# Autodesk Inventor assembly: Ring1_Assembly_JacobMorgan_030415_pd3.ipt
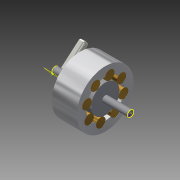
[picture p0: Inventor's stored thumbnail of the model, 180x180]
Saved by Autodesk Inventor 2015 (Build 190159000, 159)
## iProperties
Created: 2015-03-04
Part Number: Ring1_Assembly_JacobMorgan_030415_pd3.ipt
Document SubType Name: Assembly
Designer: WASHHSST
Author: WASHHSST
## Documents named in this file (6)
- E:\Ring1_Assembly_JacobMorgan_030415_pd3.ipt.iam
- E:\Ring1_NewDimensions_JacobMorgan_030215_pd3.ipt
- E:\Ring1_Center_JacobMorgan_030415_pd3.ipt
- E:\Ring1_Roller_JacobMorgan_030315_pd3.ipt
- E:\ring1_arm_JacobMorgan_030515_pd3.ipt
- E:\ring1_rollerFace_JacobMorgan_030515_pd3.ipt
## Components (19 placed, 5 different names)
1. Ring1_NewDimensions_JacobMorgan_030215_pd3:1 — Flush:1, Flush:2, Tangent:1, Flush:3, Flush:4, Flush:5, Flush:6, Flush:7, Flush:8, Flush:9, Tangent:2, Tangent:3, Tangent:4, Tangent:5, Tangent:6, Tangent:7, Tangent:8, Flush:10, Flush:11
2. Ring1_Center_JacobMorgan_030415_pd3:1 — Flush:1, Flush:2, Tangent:1, Tangent:12, Tangent:32, Tangent:33, Mate:9, Rotation:7
3. Ring1_Center_JacobMorgan_030415_pd3:2 — Flush:3, Tangent:4, Tangent:18, Tangent:26, Tangent:27, Mate:6, Rotation:2
4. Ring1_Center_JacobMorgan_030415_pd3:3 — Flush:4, Tangent:2, Tangent:10, Tangent:20, Tangent:22, Tangent:23, Mate:4, Rotation:6
5. Ring1_Center_JacobMorgan_030415_pd3:4 — Flush:5, Tangent:3, Tangent:9, Tangent:19, Rotation:1, Tangent:24, Tangent:25, Mate:5
6. Ring1_Center_JacobMorgan_030415_pd3:5 — Flush:6, Tangent:5, Tangent:17, Rotation:3, Tangent:30, Tangent:31, Mate:8
7. Ring1_Center_JacobMorgan_030415_pd3:6 — Flush:7, Tangent:8, Tangent:13, Tangent:34, Tangent:35, Mate:10, Rotation:8
8. Ring1_Center_JacobMorgan_030415_pd3:7 — Flush:8, Tangent:6, Tangent:16, Tangent:28, Tangent:29, Mate:7, Rotation:4
9. Ring1_Center_JacobMorgan_030415_pd3:8 — Flush:9, Tangent:7, Tangent:11, Flush:11, Tangent:14, Tangent:15, Tangent:36, Tangent:37, Mate:11, Rotation:5
10. Ring1_Roller_JacobMorgan_030315_pd3:1 — Flush:10, Tangent:9, Tangent:10, Tangent:11, Tangent:12, Tangent:13, Tangent:14, Tangent:15, Tangent:16, Tangent:17, Tangent:18, Tangent:19, Tangent:20, Mate:1, Mate:2, Mate:3, Tangent:21, Rotation:1, Rotation:2, Rotation:3, Rotation:4, Rotation:5, Rotation:6, Rotation:7, Rotation:8
11. ring1_arm_JacobMorgan_030515_pd3:1 — Mate:1, Mate:2, Mate:3, Tangent:21
12. ring1_rollerFace_JacobMorgan_030515_pd3:2 — Tangent:24, Tangent:25, Mate:5
13. ring1_rollerFace_JacobMorgan_030515_pd3:9 — Tangent:36, Tangent:37, Mate:11
14. ring1_rollerFace_JacobMorgan_030515_pd3:10 — Tangent:22, Tangent:23, Mate:4
15. ring1_rollerFace_JacobMorgan_030515_pd3:12 — Tangent:26, Tangent:27, Mate:6
16. ring1_rollerFace_JacobMorgan_030515_pd3:13 — Tangent:34, Tangent:35, Mate:10
17. ring1_rollerFace_JacobMorgan_030515_pd3:14 — Tangent:28, Tangent:29, Mate:7
18. ring1_rollerFace_JacobMorgan_030515_pd3:15 — Tangent:32, Tangent:33, Mate:9
19. ring1_rollerFace_JacobMorgan_030515_pd3:16 — Tangent:30, Tangent:31, Mate:8
## Relationships (67: Tangent 37, Flush 11, Mate 11, RelateRotation 8)
- Flush:1: Ring1_NewDimensions_JacobMorgan_030215_pd3:1 ↔ Ring1_Center_JacobMorgan_030415_pd3:1
- Flush:2: Ring1_NewDimensions_JacobMorgan_030215_pd3:1 ↔ Ring1_Center_JacobMorgan_030415_pd3:1
- Tangent:1: Ring1_NewDimensions_JacobMorgan_030215_pd3:1 ↔ Ring1_Center_JacobMorgan_030415_pd3:1
- Flush:3: Ring1_NewDimensions_JacobMorgan_030215_pd3:1 ↔ Ring1_Center_JacobMorgan_030415_pd3:2
- Flush:4: Ring1_NewDimensions_JacobMorgan_030215_pd3:1 ↔ Ring1_Center_JacobMorgan_030415_pd3:3
- Flush:5: Ring1_NewDimensions_JacobMorgan_030215_pd3:1 ↔ Ring1_Center_JacobMorgan_030415_pd3:4
- Flush:6: Ring1_NewDimensions_JacobMorgan_030215_pd3:1 ↔ Ring1_Center_JacobMorgan_030415_pd3:5
- Flush:7: Ring1_NewDimensions_JacobMorgan_030215_pd3:1 ↔ Ring1_Center_JacobMorgan_030415_pd3:6
- Flush:8: Ring1_NewDimensions_JacobMorgan_030215_pd3:1 ↔ Ring1_Center_JacobMorgan_030415_pd3:7
- Flush:9: Ring1_NewDimensions_JacobMorgan_030215_pd3:1 ↔ Ring1_Center_JacobMorgan_030415_pd3:8
- Tangent:2: Ring1_NewDimensions_JacobMorgan_030215_pd3:1 ↔ Ring1_Center_JacobMorgan_030415_pd3:3
- Tangent:3: Ring1_NewDimensions_JacobMorgan_030215_pd3:1 ↔ Ring1_Center_JacobMorgan_030415_pd3:4
- Tangent:4: Ring1_NewDimensions_JacobMorgan_030215_pd3:1 ↔ Ring1_Center_JacobMorgan_030415_pd3:2
- Tangent:5: Ring1_NewDimensions_JacobMorgan_030215_pd3:1 ↔ Ring1_Center_JacobMorgan_030415_pd3:5
- Tangent:6: Ring1_NewDimensions_JacobMorgan_030215_pd3:1 ↔ Ring1_Center_JacobMorgan_030415_pd3:7
- Tangent:7: Ring1_NewDimensions_JacobMorgan_030215_pd3:1 ↔ Ring1_Center_JacobMorgan_030415_pd3:8
- Tangent:8: Ring1_NewDimensions_JacobMorgan_030215_pd3:1 ↔ Ring1_Center_JacobMorgan_030415_pd3:6
- Flush:10: Ring1_NewDimensions_JacobMorgan_030215_pd3:1 ↔ Ring1_Roller_JacobMorgan_030315_pd3:1
- Tangent:9: Ring1_Center_JacobMorgan_030415_pd3:4 ↔ Ring1_Roller_JacobMorgan_030315_pd3:1
- Tangent:10: Ring1_Center_JacobMorgan_030415_pd3:3 ↔ Ring1_Roller_JacobMorgan_030315_pd3:1
- Tangent:11: Ring1_Center_JacobMorgan_030415_pd3:8 ↔ Ring1_Roller_JacobMorgan_030315_pd3:1
- Flush:11: Ring1_NewDimensions_JacobMorgan_030215_pd3:1 ↔ Ring1_Center_JacobMorgan_030415_pd3:8
- Tangent:12: Ring1_Center_JacobMorgan_030415_pd3:1 ↔ Ring1_Roller_JacobMorgan_030315_pd3:1
- Tangent:13: Ring1_Center_JacobMorgan_030415_pd3:6 ↔ Ring1_Roller_JacobMorgan_030315_pd3:1
- Tangent:14: Ring1_Center_JacobMorgan_030415_pd3:8 ↔ Ring1_Roller_JacobMorgan_030315_pd3:1
- Tangent:15: Ring1_Center_JacobMorgan_030415_pd3:8 ↔ Ring1_Roller_JacobMorgan_030315_pd3:1
- Tangent:16: Ring1_Center_JacobMorgan_030415_pd3:7 ↔ Ring1_Roller_JacobMorgan_030315_pd3:1
- Tangent:17: Ring1_Center_JacobMorgan_030415_pd3:5 ↔ Ring1_Roller_JacobMorgan_030315_pd3:1
- Tangent:18: Ring1_Center_JacobMorgan_030415_pd3:2 ↔ Ring1_Roller_JacobMorgan_030315_pd3:1
- Tangent:19: Ring1_Center_JacobMorgan_030415_pd3:4 ↔ Ring1_Roller_JacobMorgan_030315_pd3:1
- Tangent:20: Ring1_Center_JacobMorgan_030415_pd3:3 ↔ Ring1_Roller_JacobMorgan_030315_pd3:1
- Mate:1: Ring1_Roller_JacobMorgan_030315_pd3:1 ↔ ring1_arm_JacobMorgan_030515_pd3:1
- Mate:2: Ring1_Roller_JacobMorgan_030315_pd3:1 ↔ ring1_arm_JacobMorgan_030515_pd3:1
- Mate:3: Ring1_Roller_JacobMorgan_030315_pd3:1 ↔ ring1_arm_JacobMorgan_030515_pd3:1
- Tangent:21: Ring1_Roller_JacobMorgan_030315_pd3:1 ↔ ring1_arm_JacobMorgan_030515_pd3:1
- Rotation:1 [RelateRotation] (0.333 ul): Ring1_Center_JacobMorgan_030415_pd3:4 ↔ Ring1_Roller_JacobMorgan_030315_pd3:1
- Tangent:22: Ring1_Center_JacobMorgan_030415_pd3:3 ↔ ring1_rollerFace_JacobMorgan_030515_pd3:10
- Tangent:23: Ring1_Center_JacobMorgan_030415_pd3:3 ↔ ring1_rollerFace_JacobMorgan_030515_pd3:10
- Mate:4: Ring1_Center_JacobMorgan_030415_pd3:3 ↔ ring1_rollerFace_JacobMorgan_030515_pd3:10
- Tangent:24: Ring1_Center_JacobMorgan_030415_pd3:4 ↔ ring1_rollerFace_JacobMorgan_030515_pd3:2
- Tangent:25: Ring1_Center_JacobMorgan_030415_pd3:4 ↔ ring1_rollerFace_JacobMorgan_030515_pd3:2
- Mate:5: Ring1_Center_JacobMorgan_030415_pd3:4 ↔ ring1_rollerFace_JacobMorgan_030515_pd3:2
- Tangent:26: Ring1_Center_JacobMorgan_030415_pd3:2 ↔ ring1_rollerFace_JacobMorgan_030515_pd3:12
- Tangent:27: Ring1_Center_JacobMorgan_030415_pd3:2 ↔ ring1_rollerFace_JacobMorgan_030515_pd3:12
- Mate:6: Ring1_Center_JacobMorgan_030415_pd3:2 ↔ ring1_rollerFace_JacobMorgan_030515_pd3:12
- Tangent:28: Ring1_Center_JacobMorgan_030415_pd3:7 ↔ ring1_rollerFace_JacobMorgan_030515_pd3:14
- Tangent:29: Ring1_Center_JacobMorgan_030415_pd3:7 ↔ ring1_rollerFace_JacobMorgan_030515_pd3:14
- Mate:7: Ring1_Center_JacobMorgan_030415_pd3:7 ↔ ring1_rollerFace_JacobMorgan_030515_pd3:14
- Rotation:2 [RelateRotation] (0.333 ul): Ring1_Center_JacobMorgan_030415_pd3:2 ↔ Ring1_Roller_JacobMorgan_030315_pd3:1
- Rotation:3 [RelateRotation] (0.333 ul): Ring1_Center_JacobMorgan_030415_pd3:5 ↔ Ring1_Roller_JacobMorgan_030315_pd3:1
- Rotation:4 [RelateRotation] (3 ul): Ring1_Center_JacobMorgan_030415_pd3:7 ↔ Ring1_Roller_JacobMorgan_030315_pd3:1
- Tangent:30: Ring1_Center_JacobMorgan_030415_pd3:5 ↔ ring1_rollerFace_JacobMorgan_030515_pd3:16
- Tangent:31: Ring1_Center_JacobMorgan_030415_pd3:5 ↔ ring1_rollerFace_JacobMorgan_030515_pd3:16
- Mate:8: Ring1_Center_JacobMorgan_030415_pd3:5 ↔ ring1_rollerFace_JacobMorgan_030515_pd3:16
- Tangent:32: Ring1_Center_JacobMorgan_030415_pd3:1 ↔ ring1_rollerFace_JacobMorgan_030515_pd3:15
- Tangent:33: Ring1_Center_JacobMorgan_030415_pd3:1 ↔ ring1_rollerFace_JacobMorgan_030515_pd3:15
- Mate:9: Ring1_Center_JacobMorgan_030415_pd3:1 ↔ ring1_rollerFace_JacobMorgan_030515_pd3:15
- Tangent:34: Ring1_Center_JacobMorgan_030415_pd3:6 ↔ ring1_rollerFace_JacobMorgan_030515_pd3:13
- Tangent:35: Ring1_Center_JacobMorgan_030415_pd3:6 ↔ ring1_rollerFace_JacobMorgan_030515_pd3:13
- Mate:10: Ring1_Center_JacobMorgan_030415_pd3:6 ↔ ring1_rollerFace_JacobMorgan_030515_pd3:13
- Tangent:36: Ring1_Center_JacobMorgan_030415_pd3:8 ↔ ring1_rollerFace_JacobMorgan_030515_pd3:9
- Tangent:37: Ring1_Center_JacobMorgan_030415_pd3:8 ↔ ring1_rollerFace_JacobMorgan_030515_pd3:9
- Mate:11: Ring1_Center_JacobMorgan_030415_pd3:8 ↔ ring1_rollerFace_JacobMorgan_030515_pd3:9
- Rotation:5 [RelateRotation] (3 ul): Ring1_Center_JacobMorgan_030415_pd3:8 ↔ Ring1_Roller_JacobMorgan_030315_pd3:1
- Rotation:6 [RelateRotation] (0.333 ul): Ring1_Center_JacobMorgan_030415_pd3:3 ↔ Ring1_Roller_JacobMorgan_030315_pd3:1
- Rotation:7 [RelateRotation] (3 ul): Ring1_Center_JacobMorgan_030415_pd3:1 ↔ Ring1_Roller_JacobMorgan_030315_pd3:1
- Rotation:8 [RelateRotation] (3 ul): Ring1_Center_JacobMorgan_030415_pd3:6 ↔ Ring1_Roller_JacobMorgan_030315_pd3:1
